# Autodesk Inventor assembly: Box_Assembly
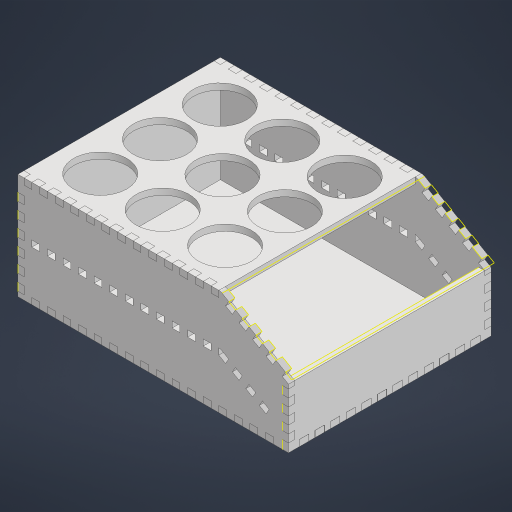
[picture p0: Inventor's stored thumbnail of the model, 512x512]
Saved by Autodesk Inventor 2023 (Build 270158030, 158C)
## iProperties
Created: 2022-06-21
Part Number: Box_Assembly
Document SubType Name: Assembly
Designer: Simon
Author: Simon
## Documents named in this file (6)
- C:\Users\simfe\Desktop\2.Semester\Technische Grundlagen-II\Pixie\3d-modelle\.iam's\Box_Assembly.iam
- C:\Users\simfe\Desktop\2.Semester\Technische Grundlagen-II\Pixie\3d-modelle\.ipt's\SeitenWand.ipt
- C:\Users\simfe\Desktop\2.Semester\Technische Grundlagen-II\Pixie\3d-modelle\.ipt's\BodenWand.ipt
- C:\Users\simfe\Desktop\2.Semester\Technische Grundlagen-II\Pixie\3d-modelle\.ipt's\VorderWand.ipt
- C:\Users\simfe\Desktop\2.Semester\Technische Grundlagen-II\Pixie\3d-modelle\.ipt's\BackWand.ipt
- C:\Users\simfe\Desktop\2.Semester\Technische Grundlagen-II\Pixie\3d-modelle\.ipt's\Top cover with groves.ipt
## Components (6 placed, 5 different names)
1. SeitenWand:1 — Mate:1, Flush:1, Flush:2, Mate:5, Mate:9, Mate:10, Mate:13
2. SeitenWand:2 — Mate:1, Flush:1, Flush:2, Mate:2, Mate:3, Mate:4, Mate:6, Mate:12
3. BodenWand:1 — Mate:2, Mate:3, Mate:4, Mate:7, Mate:8
4. VorderWand:1 — Mate:5, Mate:6, Mate:7
5. BackWand:1 — Mate:8, Mate:9, Mate:10, Mate:11
6. Top cover with groves:1 — Mate:11, Mate:12, Mate:13
## Relationships (15: Mate 13, Flush 2)
- Mate:1 (122 mm): SeitenWand:1 ↔ SeitenWand:2
- Flush:1: SeitenWand:1 ↔ SeitenWand:2
- Flush:2: SeitenWand:1 ↔ SeitenWand:2
- Mate:2: SeitenWand:2 ↔ BodenWand:1
- Mate:3: SeitenWand:2 ↔ BodenWand:1
- Mate:4: SeitenWand:2 ↔ BodenWand:1
- Mate:5: SeitenWand:1 ↔ VorderWand:1
- Mate:6: SeitenWand:2 ↔ VorderWand:1
- Mate:7: BodenWand:1 ↔ VorderWand:1
- Mate:8: BodenWand:1 ↔ BackWand:1
- Mate:9: SeitenWand:1 ↔ BackWand:1
- Mate:10: SeitenWand:1 ↔ BackWand:1
- Mate:11: BackWand:1 ↔ Top cover with groves:1
- Mate:12: SeitenWand:2 ↔ Top cover with groves:1
- Mate:13: SeitenWand:1 ↔ Top cover with groves:1
